# Autodesk Inventor assembly: Custom_Delta_Assembly
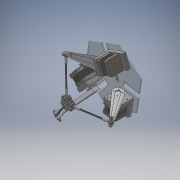
[picture p0: Inventor's stored thumbnail of the model, 180x180]
Saved by Autodesk Inventor 2019 (Build 230136000, 136)
## iProperties
Created: 2019-07-06
Part Number: Custom_Delta_Assembly
Document SubType Name: Assembly
Designer: Jorian Brusind
Author: Jorian Brusind
## Documents named in this file (11)
- C:\Users\Jorian Brusind\Documents\GitHub\ECE44x_Senior_Design\Design files\Delta Robot Arm\Inventor Files\Custom_Delta\Custom_Delta_Assembly.iam
- C:\Users\Jorian Brusind\Documents\GitHub\ECE44x_Senior_Design\Design files\Delta Robot Arm\Inventor Files\Custom_Delta\Stepper_Face.ipt
- C:\Users\Jorian Brusind\Documents\GitHub\ECE44x_Senior_Design\Design files\Delta Robot Arm\Inventor Files\nema-17-stepper-motor-with-v2-damper-1.snapshot.3\Nema 17  Stepper Motor length 34mm.ipt
- C:\Users\Jorian Brusind\Documents\GitHub\ECE44x_Senior_Design\Design files\Delta Robot Arm\Inventor Files\Stepper_Collar\products\12488\step\model.ipt
- C:\Users\Jorian Brusind\Documents\GitHub\ECE44x_Senior_Design\Design files\Delta Robot Arm\Inventor Files\Custom_Delta\Delta_Arm.ipt
- C:\Users\Jorian Brusind\Documents\GitHub\ECE44x_Senior_Design\Design files\Delta Robot Arm\Inventor Files\Custom_Delta\Delta_Top.ipt
- C:\Users\Jorian Brusind\Documents\GitHub\ECE44x_Senior_Design\Design files\Delta Robot Arm\Inventor Files\McMaster Files\59935K140_METRIC BALL JOINT ROD END.ipt
- C:\Users\Jorian Brusind\Documents\GitHub\ECE44x_Senior_Design\Design files\Delta Robot Arm\Inventor Files\Metric nuts\Nut M4.ipt
- C:\Users\Jorian Brusind\Documents\GitHub\ECE44x_Senior_Design\Design files\Delta Robot Arm\Inventor Files\McMaster Files\94595A216_LOW-STRENGTH ZINC-PLATED STEEL THREADED ROD.ipt
- C:\Users\Jorian Brusind\Documents\GitHub\ECE44x_Senior_Design\Design files\Delta Robot Arm\Inventor Files\Metric bolt\Bolt M4 25mm.ipt
- C:\Users\Jorian Brusind\Documents\GitHub\ECE44x_Senior_Design\Design files\Delta Robot Arm\Inventor Files\Custom_Delta\Custom_Delta_End_Effector.ipt
## Components (33 placed, 10 different names)
1. Stepper_Face:1 — Mate:1, Mate:2, Mate:3, Mate:27, Mate:28, Mate:29
2. Nema 17  Stepper Motor length 34mm:1 — Mate:1, Mate:2, Mate:3, Mate:4, Flush:1
3. model:1 — Mate:4, Flush:1, Mate:7, Mate:8, Mate:9
4. Delta_Arm:1 — Mate:7, Mate:8, Flush:2, Mate:9, Mate:33, Mate:78
5. Stepper_Face:2 — Mate:30, Mate:31, Mate:32
6. Nema 17  Stepper Motor length 34mm:2
7. model:2
8. Delta_Arm:2 — Mate:44, Mate:73, Mate:74, Mate:75, Mate:77
9. Stepper_Face:3 — Mate:24, Mate:25, Mate:26
10. Nema 17  Stepper Motor length 34mm:3
11. model:3
12. Delta_Arm:3 — Mate:72, Mate:83, Mate:84, Mate:86, Mate:87
13. Delta_Top:1 — Mate:24, Mate:25, Mate:26, Mate:27, Mate:28, Mate:29, Mate:30, Mate:31, Mate:32, Mate:104
14. 59935K140_METRIC BALL JOINT ROD END:2 — Mate:33, Mate:64, Mate:70, Mate:78
15. 59935K140_METRIC BALL JOINT ROD END:3 — Mate:44, Mate:62, Mate:66, Mate:73
16. 59935K140_METRIC BALL JOINT ROD END:5 — Mate:59, Mate:60, Mate:72, Mate:83
17. 94595A216_LOW-STRENGTH ZINC-PLATED STEEL THREADED ROD:1 — Mate:64, Mate:70, Mate:90, Mate:93
18. 94595A216_LOW-STRENGTH ZINC-PLATED STEEL THREADED ROD:5 — Mate:62, Mate:66, Mate:89, Mate:91
19. 94595A216_LOW-STRENGTH ZINC-PLATED STEEL THREADED ROD:6 — Mate:59, Mate:60, Mate:88, Mate:92
20. Bolt M4 25mm:1 — Mate:74, Mate:75, Mate:76
21. Bolt M4 25mm:3 — Mate:84, Mate:85, Mate:86
22. Nut M4:2 — Mate:76, Mate:77
23. Nut M4:3 — Mate:85, Mate:87
24. 59935K140_METRIC BALL JOINT ROD END:6 — Mate:88, Mate:92, Mate:98, Mate:99
25. 59935K140_METRIC BALL JOINT ROD END:7 — Mate:89, Mate:91, Mate:102, Mate:103
26. 59935K140_METRIC BALL JOINT ROD END:8 — Mate:90, Mate:93, Mate:100, Mate:101, Mate:105
27. Custom_Delta_End_Effector:1 — Mate:98, Mate:99, Mate:100, Mate:101, Mate:102, Mate:103, Mate:104, Mate:106, Mate:107, Mate:108, Mate:109, Mate:110, Mate:114, Mate:115, Mate:116
28. Bolt M4 25mm:4 — Mate:105, Mate:110, Mate:113
29. Bolt M4 25mm:5 — Mate:106, Mate:109, Mate:111
30. Bolt M4 25mm:6 — Mate:107, Mate:108, Mate:112
31. Nut M4:4 — Mate:111, Mate:115
32. Nut M4:5 — Mate:112, Mate:114
33. Nut M4:6 — Mate:113, Mate:116
## Relationships (79: Mate 75, Flush 4)
- Mate:1: Stepper_Face:1 ↔ Nema 17  Stepper Motor length 34mm:1
- Mate:2: Stepper_Face:1 ↔ Nema 17  Stepper Motor length 34mm:1
- Mate:3: Stepper_Face:1 ↔ Nema 17  Stepper Motor length 34mm:1
- Mate:4: Nema 17  Stepper Motor length 34mm:1 ↔ model:1
- Flush:1: Nema 17  Stepper Motor length 34mm:1 ↔ model:1
- Mate:7: model:1 ↔ Delta_Arm:1
- Mate:8: model:1 ↔ Delta_Arm:1
- Flush:2: Delta_Arm:1
- Mate:9: model:1 ↔ Delta_Arm:1
- [Mate]: Stepper_Face:2 ↔ Nema 17  Stepper Motor length 34mm:2
- [Mate]: Stepper_Face:2 ↔ Nema 17  Stepper Motor length 34mm:2
- [Mate]: Stepper_Face:2 ↔ Nema 17  Stepper Motor length 34mm:2
- [Mate]: Nema 17  Stepper Motor length 34mm:2 ↔ model:2
- [Flush]: Nema 17  Stepper Motor length 34mm:2 ↔ model:2
- [Mate]: model:2 ↔ Delta_Arm:2
- [Mate]: model:2 ↔ Delta_Arm:2
- [Mate]: model:2 ↔ Delta_Arm:2
- [Mate]: Stepper_Face:3 ↔ Nema 17  Stepper Motor length 34mm:3
- [Mate]: Stepper_Face:3 ↔ Nema 17  Stepper Motor length 34mm:3
- [Mate]: Stepper_Face:3 ↔ Nema 17  Stepper Motor length 34mm:3
- [Mate]: Nema 17  Stepper Motor length 34mm:3 ↔ model:3
- [Flush]: Nema 17  Stepper Motor length 34mm:3 ↔ model:3
- [Mate]: model:3 ↔ Delta_Arm:3
- [Mate]: model:3 ↔ Delta_Arm:3
- [Mate]: model:3 ↔ Delta_Arm:3
- Mate:24: Stepper_Face:3 ↔ Delta_Top:1
- Mate:25: Stepper_Face:3 ↔ Delta_Top:1
- Mate:26: Stepper_Face:3 ↔ Delta_Top:1
- Mate:27: Stepper_Face:1 ↔ Delta_Top:1
- Mate:28: Stepper_Face:1 ↔ Delta_Top:1
- Mate:29: Stepper_Face:1 ↔ Delta_Top:1
- Mate:30: Stepper_Face:2 ↔ Delta_Top:1
- Mate:31: Stepper_Face:2 ↔ Delta_Top:1
- Mate:32: Stepper_Face:2 ↔ Delta_Top:1
- Mate:33: Delta_Arm:1 ↔ 59935K140_METRIC BALL JOINT ROD END:2
- Mate:44: Delta_Arm:2 ↔ 59935K140_METRIC BALL JOINT ROD END:3
- Mate:59: 59935K140_METRIC BALL JOINT ROD END:5 ↔ 94595A216_LOW-STRENGTH ZINC-PLATED STEEL THREADED ROD:6
- Mate:60: 59935K140_METRIC BALL JOINT ROD END:5 ↔ 94595A216_LOW-STRENGTH ZINC-PLATED STEEL THREADED ROD:6
- Mate:62: 59935K140_METRIC BALL JOINT ROD END:3 ↔ 94595A216_LOW-STRENGTH ZINC-PLATED STEEL THREADED ROD:5
- Mate:64: 59935K140_METRIC BALL JOINT ROD END:2 ↔ 94595A216_LOW-STRENGTH ZINC-PLATED STEEL THREADED ROD:1
- Mate:66: 59935K140_METRIC BALL JOINT ROD END:3 ↔ 94595A216_LOW-STRENGTH ZINC-PLATED STEEL THREADED ROD:5
- Mate:70: 59935K140_METRIC BALL JOINT ROD END:2 ↔ 94595A216_LOW-STRENGTH ZINC-PLATED STEEL THREADED ROD:1
- Mate:72: Delta_Arm:3 ↔ 59935K140_METRIC BALL JOINT ROD END:5
- Mate:73 (0.55 mm): Delta_Arm:2 ↔ 59935K140_METRIC BALL JOINT ROD END:3
- Mate:74: Delta_Arm:2 ↔ Bolt M4 25mm:1
- Mate:75: Delta_Arm:2 ↔ Bolt M4 25mm:1
- Mate:76: Bolt M4 25mm:1 ↔ Nut M4:2
- Mate:77: Delta_Arm:2 ↔ Nut M4:2
- Mate:78 (0.55 mm): Delta_Arm:1 ↔ 59935K140_METRIC BALL JOINT ROD END:2
- Mate:83 (0.55 mm): Delta_Arm:3 ↔ 59935K140_METRIC BALL JOINT ROD END:5
- Mate:84: Delta_Arm:3 ↔ Bolt M4 25mm:3
- Mate:85: Bolt M4 25mm:3 ↔ Nut M4:3
- Mate:86: Delta_Arm:3 ↔ Bolt M4 25mm:3
- Mate:87: Delta_Arm:3 ↔ Nut M4:3
- Mate:88: 94595A216_LOW-STRENGTH ZINC-PLATED STEEL THREADED ROD:6 ↔ 59935K140_METRIC BALL JOINT ROD END:6
- Mate:89: 94595A216_LOW-STRENGTH ZINC-PLATED STEEL THREADED ROD:5 ↔ 59935K140_METRIC BALL JOINT ROD END:7
- Mate:90: 94595A216_LOW-STRENGTH ZINC-PLATED STEEL THREADED ROD:1 ↔ 59935K140_METRIC BALL JOINT ROD END:8
- Mate:91: 94595A216_LOW-STRENGTH ZINC-PLATED STEEL THREADED ROD:5 ↔ 59935K140_METRIC BALL JOINT ROD END:7
- Mate:92: 94595A216_LOW-STRENGTH ZINC-PLATED STEEL THREADED ROD:6 ↔ 59935K140_METRIC BALL JOINT ROD END:6
- Mate:93: 94595A216_LOW-STRENGTH ZINC-PLATED STEEL THREADED ROD:1 ↔ 59935K140_METRIC BALL JOINT ROD END:8
- Mate:98: 59935K140_METRIC BALL JOINT ROD END:6 ↔ Custom_Delta_End_Effector:1
- Mate:99 (0.55 mm): 59935K140_METRIC BALL JOINT ROD END:6 ↔ Custom_Delta_End_Effector:1
- Mate:100: 59935K140_METRIC BALL JOINT ROD END:8 ↔ Custom_Delta_End_Effector:1
- Mate:101 (0.55 mm): 59935K140_METRIC BALL JOINT ROD END:8 ↔ Custom_Delta_End_Effector:1
- Mate:102: 59935K140_METRIC BALL JOINT ROD END:7 ↔ Custom_Delta_End_Effector:1
- Mate:103 (0.55 mm): 59935K140_METRIC BALL JOINT ROD END:7 ↔ Custom_Delta_End_Effector:1
- Mate:104: Delta_Top:1 ↔ Custom_Delta_End_Effector:1
- Mate:105: 59935K140_METRIC BALL JOINT ROD END:8 ↔ Bolt M4 25mm:4
- Mate:106: Custom_Delta_End_Effector:1 ↔ Bolt M4 25mm:5
- Mate:107: Custom_Delta_End_Effector:1 ↔ Bolt M4 25mm:6
- Mate:108: Custom_Delta_End_Effector:1 ↔ Bolt M4 25mm:6
- Mate:109: Custom_Delta_End_Effector:1 ↔ Bolt M4 25mm:5
- Mate:110: Custom_Delta_End_Effector:1 ↔ Bolt M4 25mm:4
- Mate:111: Bolt M4 25mm:5 ↔ Nut M4:4
- Mate:112: Bolt M4 25mm:6 ↔ Nut M4:5
- Mate:113: Bolt M4 25mm:4 ↔ Nut M4:6
- Mate:114: Custom_Delta_End_Effector:1 ↔ Nut M4:5
- Mate:115: Custom_Delta_End_Effector:1 ↔ Nut M4:4
- Mate:116: Custom_Delta_End_Effector:1 ↔ Nut M4:6
## Named parameters: d13_d12 = 0 mm, d14_d5 = 0 mm, d15_d7 = 0 mm, d16_d8 = 0 mm, d17_d0 = 0 mm, d18_d1 = 0 mm, d19_d2 = 0 mm, d20_d3 = 0 mm, d21_d12 = 0 mm, d22_d5 = 0 mm, d23_d7 = 0 mm, d24_d8 = 0 mm, d25_d0 = 0 mm, d26_d1 = 0 mm, d27_d2 = 0 mm, d28_d3 = 0 mm
